# Autodesk Inventor assembly: Arduino Nano V3 assemble
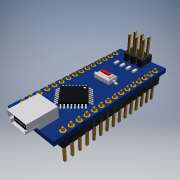
[picture p0: Inventor's stored thumbnail of the model, 180x180]
Saved by Autodesk Inventor 2017 (Build 210142000, 142)
## iProperties
Created: 2017-09-09
Part Number: Arduino Nano V3 assemble
Document SubType Name: Assembly
Designer: denoqs
Author: denoqs
## Documents named in this file (4)
- E:\Graphic Development\Autodesk Inventor\Inventor output\Arduino things\Arduino Nano V3 assemble.iam
- E:\Graphic Development\Autodesk Inventor\Inventor output\Arduino things\Arduino Nano V3 PCB.ipt
- E:\Graphic Development\Autodesk Inventor\Inventor output\Arduino things\Arduino header\Male straight header 15p.iam
- E:\Graphic Development\Autodesk Inventor\Inventor output\Arduino things\Arduino header\Male straight header 3p.iam
## Components (5 placed, 3 different names)
1. Arduino Nano V3 PCB:1 — Flush:1, Flush:2, Flush:3, Mate:1, Mate:2, Mate:3, Mate:4, Mate:5, Mate:6, Mate:7, Mate:8, Mate:9, Mate:10, Mate:11, Mate:12
2. Male straight header 15p:1 [sub-assembly] — Mate:1, Mate:2, Mate:3
3. Male straight header 15p:2 [sub-assembly] — Mate:4, Mate:5, Mate:6
4. Male straight header 3p:1 [sub-assembly] — Mate:7, Mate:8, Mate:9
5. Male straight header 3p:2 [sub-assembly] — Mate:10, Mate:11, Mate:12
## Relationships (15: Mate 12, Flush 3)
- Flush:1: Arduino Nano V3 PCB:1
- Flush:2: Arduino Nano V3 PCB:1
- Flush:3: Arduino Nano V3 PCB:1
- Mate:1: Arduino Nano V3 PCB:1 ↔ Male straight header 15p:1
- Mate:2: Arduino Nano V3 PCB:1 ↔ Male straight header 15p:1
- Mate:3: Arduino Nano V3 PCB:1 ↔ Male straight header 15p:1
- Mate:4: Arduino Nano V3 PCB:1 ↔ Male straight header 15p:2
- Mate:5: Arduino Nano V3 PCB:1 ↔ Male straight header 15p:2
- Mate:6: Arduino Nano V3 PCB:1 ↔ Male straight header 15p:2
- Mate:7: Arduino Nano V3 PCB:1 ↔ Male straight header 3p:1
- Mate:8: Arduino Nano V3 PCB:1 ↔ Male straight header 3p:1
- Mate:9: Arduino Nano V3 PCB:1 ↔ Male straight header 3p:1
- Mate:10: Arduino Nano V3 PCB:1 ↔ Male straight header 3p:2
- Mate:11: Arduino Nano V3 PCB:1 ↔ Male straight header 3p:2
- Mate:12: Arduino Nano V3 PCB:1 ↔ Male straight header 3p:2
